# Autodesk Inventor assembly: PinecilCaseASM
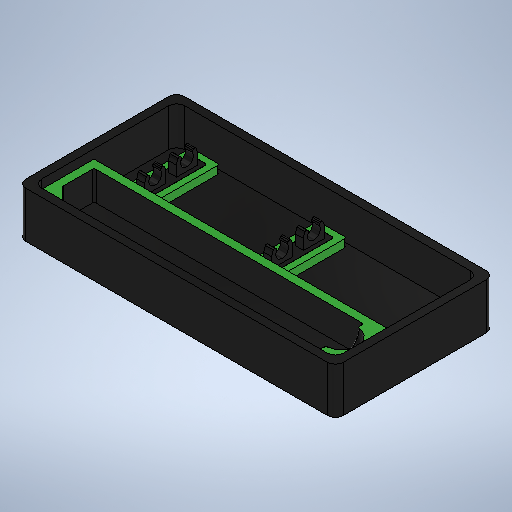
[picture p0: Inventor's stored thumbnail of the model, 512x512]
Saved by Autodesk Inventor 2026 (Build 300175050, 175E)
## iProperties
Created: 2025-10-09
Part Number: PinecilCaseASM
Document SubType Name: Assembly
Designer: Nicholas M
Author: Nicholas M
## Documents named in this file (3)
- C:\Users\nmari\OneDrive\Documents\Inventor Parts\Pinecil Case\PinecilCaseASM.iam
- C:\Users\nmari\OneDrive\Documents\Inventor Parts\Pinecil Case\PinecilCaseBottom.ipt
- C:\Users\nmari\OneDrive\Documents\Inventor Parts\Pinecil Case\Pinecil Clip.ipt
## Components (3 placed, 2 different names)
1. PinecilCaseBottom:1 — Rigid:1, Rigid:2
2. Pinecil Clip:1 — Rigid:1
3. Pinecil Clip:2 — Rigid:2
## Relationships (2: WeldJoint 2)
- Rigid:1 [WeldJoint]: PinecilCaseBottom:1 ↔ Pinecil Clip:1
- Rigid:2 [WeldJoint]: PinecilCaseBottom:1 ↔ Pinecil Clip:2
